# Autodesk Inventor assembly: wozek
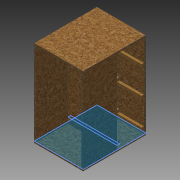
[picture p0: Inventor's stored thumbnail of the model, 180x180]
Saved by Autodesk Inventor 2013 (Build 170138000, 138)
## iProperties
Created: 2014-04-27
Part Number: wozek
Document SubType Name: Assembly
Designer: Masta
Author: Masta
## Documents named in this file (8)
- D:\prusa i3\assembly\szafka\wozek.iam
- D:\prusa i3\assembly\szafka\rolka_meblowa_16mm.ipt
- D:\prusa i3\assembly\szafka\wozek_podstawa.ipt
- D:\prusa i3\assembly\szafka\wozek-tyl.ipt
- D:\prusa i3\assembly\szafka\wozek_gora.ipt
- D:\prusa i3\assembly\szafka\wozek-przegroda.ipt
- D:\prusa i3\assembly\szafka\wozek-bok.ipt
- D:\prusa i3\assembly\szafka\wozek-listwa_do_szpulek.ipt
## Components (18 placed, 7 different names)
1. wozek_podstawa:1 — Insert:1, Insert:2, Insert:3, Insert:4, Insert:5, Insert:6, Insert:7, Insert:8, Insert:9, Insert:10, Insert:11, Insert:12, Mate:1, Flush:1, Flush:2, Mate:5, Mate:7, Flush:6, Flush:7, Mate:10, Flush:9, Mate:12
2. rolka_meblowa_16mm:1 — Insert:3, Insert:6
3. rolka_meblowa_16mm:2 — Insert:2, Insert:4
4. rolka_meblowa_16mm:3 — Insert:1, Insert:5
5. rolka_meblowa_16mm:4 — Insert:9, Insert:12
6. rolka_meblowa_16mm:5 — Insert:7, Insert:10
7. rolka_meblowa_16mm:6 — Insert:8, Insert:11
8. wozek-tyl:1 — Mate:1, Flush:1, Flush:2, Flush:4, Mate:4, Flush:5
9. wozek_gora:1 — Flush:4, Mate:4, Flush:5
10. wozek-przegroda:1 — Mate:5, Mate:8, Flush:8, Mate:9, Mate:11
11. wozek-bok:1 — Mate:7, Flush:6, Flush:7, Mate:8, Flush:8
12. wozek-bok:2 — Mate:9, Mate:10, Flush:9, Flush:10
13. wozek-listwa_do_szpulek:1 — Mate:11, Flush:10, Mate:12
14. wozek-listwa_do_szpulek:2
15. wozek-listwa_do_szpulek:3
16. wozek-listwa_do_szpulek:4
17. wozek-listwa_do_szpulek:5
18. wozek-listwa_do_szpulek:6
## Component patterns: (6 elements, first: wozek-listwa_do_szpulek:1)
## Relationships (30: Insert 12, Mate 9, Flush 9)
- Insert:1: wozek_podstawa:1 ↔ rolka_meblowa_16mm:3
- Insert:2: wozek_podstawa:1 ↔ rolka_meblowa_16mm:2
- Insert:3: wozek_podstawa:1 ↔ rolka_meblowa_16mm:1
- Insert:4: wozek_podstawa:1 ↔ rolka_meblowa_16mm:2
- Insert:5: wozek_podstawa:1 ↔ rolka_meblowa_16mm:3
- Insert:6: wozek_podstawa:1 ↔ rolka_meblowa_16mm:1
- Insert:7: wozek_podstawa:1 ↔ rolka_meblowa_16mm:5
- Insert:8: wozek_podstawa:1 ↔ rolka_meblowa_16mm:6
- Insert:9: wozek_podstawa:1 ↔ rolka_meblowa_16mm:4
- Insert:10: wozek_podstawa:1 ↔ rolka_meblowa_16mm:5
- Insert:11: wozek_podstawa:1 ↔ rolka_meblowa_16mm:6
- Insert:12: wozek_podstawa:1 ↔ rolka_meblowa_16mm:4
- Mate:1: wozek_podstawa:1 ↔ wozek-tyl:1
- Flush:1: wozek_podstawa:1 ↔ wozek-tyl:1
- Flush:2: wozek_podstawa:1 ↔ wozek-tyl:1
- Flush:4: wozek-tyl:1 ↔ wozek_gora:1
- Mate:4: wozek-tyl:1 ↔ wozek_gora:1
- Flush:5: wozek-tyl:1 ↔ wozek_gora:1
- Mate:5: wozek_podstawa:1 ↔ wozek-przegroda:1
- Mate:7: wozek_podstawa:1 ↔ wozek-bok:1
- Flush:6: wozek_podstawa:1 ↔ wozek-bok:1
- Flush:7: wozek_podstawa:1 ↔ wozek-bok:1
- Mate:8: wozek-przegroda:1 ↔ wozek-bok:1
- Flush:8: wozek-przegroda:1 ↔ wozek-bok:1
- Mate:9: wozek-przegroda:1 ↔ wozek-bok:2
- Mate:10: wozek_podstawa:1 ↔ wozek-bok:2
- Flush:9: wozek_podstawa:1 ↔ wozek-bok:2
- Mate:11: wozek-przegroda:1 ↔ wozek-listwa_do_szpulek:1
- Flush:10: wozek-bok:2 ↔ wozek-listwa_do_szpulek:1
- Mate:12 (45 mm): wozek_podstawa:1 ↔ wozek-listwa_do_szpulek:1
